# Autodesk Inventor assembly: Assembly1
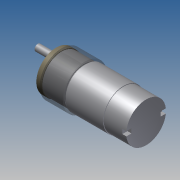
[picture p0: Inventor's stored thumbnail of the model, 180x180]
Saved by Autodesk Inventor 2012 SP1 (Build 160190100, 190)
## iProperties
Created: 2012-06-21
Part Number: Assembly1
Document SubType Name: Assembly
Designer: sta
Author: sta
## Documents named in this file (4)
- R:\Modules\SI\204_PR1 (Kart)\2012\CAD Parts\Motors\assembly moteur dentr.iam
- Y:\sta\Projet Septembre\Modellfahrzeug\2012\Adaptateur_Moteur.ipt
- Y:\sta\Projet Septembre\Modellfahrzeug\2012\Moteur.ipt
- Y:\sta\Projet Septembre\Modellfahrzeug\2012\ProtectionReducteur.ipt
## Components (3 placed, 3 different names)
1. Adaptateur_Moteur:1 — Insert:1, Mate:1, Insert:2
2. Moteur:1 — Insert:1, Mate:1
3. ProtectionReducteur:1 — Insert:2
## Relationships (3: Insert 2, Mate 1)
- Insert:1: Adaptateur_Moteur:1 ↔ Moteur:1
- Mate:1: Adaptateur_Moteur:1 ↔ Moteur:1
- Insert:2: Adaptateur_Moteur:1 ↔ ProtectionReducteur:1
